# Autodesk Inventor assembly: test_stand_cable_pose_configuration
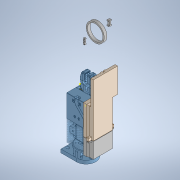
[picture p0: Inventor's stored thumbnail of the model, 180x180]
Saved by Autodesk Inventor 2022 (Build 260153000, 153)
## iProperties
Created: 2022-03-16
Part Number: test_stand_cable_pose_configuration
Document SubType Name: Assembly
Designer: kylem
Author: kylem
## Documents named in this file (7)
- C:\Users\kylem\OneDrive\Documents\GitHub\IMML_Contactile_Gripper_Hardware\test_stand\test_stand_cable_pose_configuration.iam
- C:\Users\kylem\OneDrive\Documents\GitHub\IMML_Contactile_Gripper_Hardware\Gripper_Design_NonCompliant_No_UR5.iam
- C:\Users\kylem\OneDrive\Documents\GitHub\IMML_Contactile_Gripper_Hardware\test_stand\cable_jig_base.ipt
- C:\Users\kylem\OneDrive\Documents\GitHub\IMML_Contactile_Gripper_Hardware\test_stand\cable_jig_clamp.ipt
- C:\Users\kylem\OneDrive\Documents\GitHub\IMML_Contactile_Gripper_Hardware\test_stand\cable_jig_holder_v0.ipt
- C:\Users\kylem\OneDrive\Documents\GitHub\IMML_Contactile_Gripper_Hardware\test_stand\cable_jig_lock.ipt
- C:\Users\kylem\OneDrive\Documents\GitHub\IMML_Contactile_Gripper_Hardware\test_stand\cable_jig_base_back.ipt
## Components (6 placed, 6 different names)
1. Gripper_Design_NonCompliant_No_UR5:1 [sub-assembly] — Mate:1, Mate:2, Mate:3, Mate:4, Mate:5, Mate:6
2. cable_jig_base:1 — Mate:1, Mate:2, Mate:3
3. cable_jig_clamp:1
4. cable_jig_holder_v0:1
5. cable_jig_lock:1
6. cable_jig_base_back:1 — Mate:4, Mate:5, Mate:6
## Relationships (6: Mate 6)
- Mate:1: Gripper_Design_NonCompliant_No_UR5:1 ↔ cable_jig_base:1
- Mate:2 (0.125 mm): Gripper_Design_NonCompliant_No_UR5:1 ↔ cable_jig_base:1
- Mate:3: Gripper_Design_NonCompliant_No_UR5:1 ↔ cable_jig_base:1
- Mate:4: Gripper_Design_NonCompliant_No_UR5:1 ↔ cable_jig_base_back:1
- Mate:5 (0.125 mm): Gripper_Design_NonCompliant_No_UR5:1 ↔ cable_jig_base_back:1
- Mate:6: Gripper_Design_NonCompliant_No_UR5:1 ↔ cable_jig_base_back:1
